# Autodesk Inventor assembly: Male straight header 3p
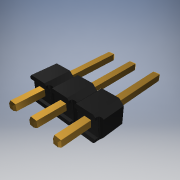
[picture p0: Inventor's stored thumbnail of the model, 180x180]
Saved by Autodesk Inventor 2017 (Build 210142000, 142)
## iProperties
Created: 2017-09-07
Part Number: Male straight header 3p
Document SubType Name: Assembly
Designer: denoqs
Author: denoqs
## Documents named in this file (3)
- E:\Graphic Development\Autodesk Inventor\Inventor output\Arduino things\Arduino header\Male straight header 3p.iam
- E:\Graphic Development\Autodesk Inventor\Inventor output\Arduino things\Arduino header\Housing male header - single.ipt
- E:\Graphic Development\Autodesk Inventor\Inventor output\Arduino things\Arduino header\Pin male header straight - single.ipt
## Components (6 placed, 2 different names)
1. Housing male header - single:1 — Flush:1, Flush:2, Flush:3, Mate:1, Mate:2, Flush:4
2. Pin male header straight - single:1 — Mate:1, Mate:2, Flush:4
3. Housing male header - single:2
4. Pin male header straight - single:2
5. Housing male header - single:3
6. Pin male header straight - single:3
## Component patterns: (3 elements, first: Housing male header - single:1 + Pin male header straight - single:1)
## Relationships (6: Flush 4, Mate 2)
- Flush:1: Housing male header - single:1
- Flush:2: Housing male header - single:1
- Flush:3: Housing male header - single:1
- Mate:1: Housing male header - single:1 ↔ Pin male header straight - single:1
- Mate:2: Housing male header - single:1 ↔ Pin male header straight - single:1
- Flush:4 (-2.54 mm): Housing male header - single:1 ↔ Pin male header straight - single:1
